# Autodesk Inventor assembly: IMU+Mag
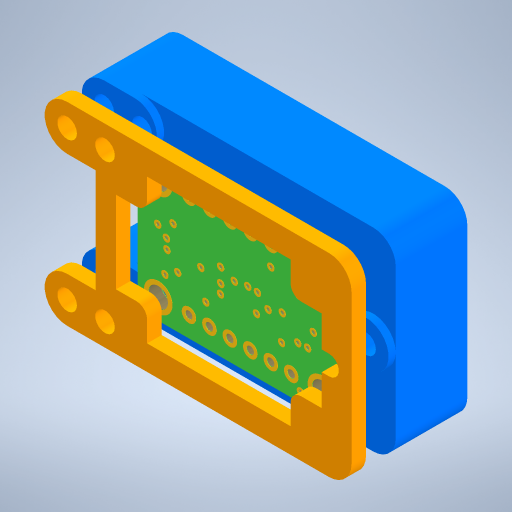
[picture p0: Inventor's stored thumbnail of the model, 512x512]
Saved by Autodesk Inventor 2023 (Build 270158000, 158)
## iProperties
Created: 2022-07-03
Part Number: IMU+Mag
Document SubType Name: Assembly
Designer: Jochen Alt
Author: Jochen Alt
## Documents named in this file (4)
- D:\Projects\Lisbeth\CAD\Common\Accessories\IMU+Mag.iam
- D:\Projects\Lisbeth\CAD\Common\Accessories\Lord Microstrain 3DM-CX5 OEM.ipt
- D:\Projects\Lisbeth\CAD\Common\Accessories\Adafruit LIS3MDL + LSM6DSOX.iam
- D:\Projects\Lisbeth\CAD\Common\Accessories\IMU Holder.ipt
## Components (3 placed, 3 different names)
1. Lord Microstrain IMU OEM:1 — Mate:2, Mate:3, Mate:4
2. Adafruit LIS3MDL + LSM6DSOX:1 [sub-assembly] — Mate:5, Angle:1, Mate:6
3. IMU Holder:1 — Mate:2, Mate:3, Mate:4, Mate:5, Angle:1, Mate:6
## Relationships (6: Mate 5, Angle 1)
- Mate:2: Lord Microstrain IMU OEM:1 ↔ IMU Holder:1
- Mate:3: Lord Microstrain IMU OEM:1 ↔ IMU Holder:1
- Mate:4: Lord Microstrain IMU OEM:1 ↔ IMU Holder:1
- Mate:5: Adafruit LIS3MDL + LSM6DSOX:1 ↔ IMU Holder:1
- Angle:1 (0 deg): Adafruit LIS3MDL + LSM6DSOX:1 ↔ IMU Holder:1
- Mate:6: Adafruit LIS3MDL + LSM6DSOX:1 ↔ IMU Holder:1
